# Autodesk Inventor assembly: 11_outer_carriage_with_cable_roller
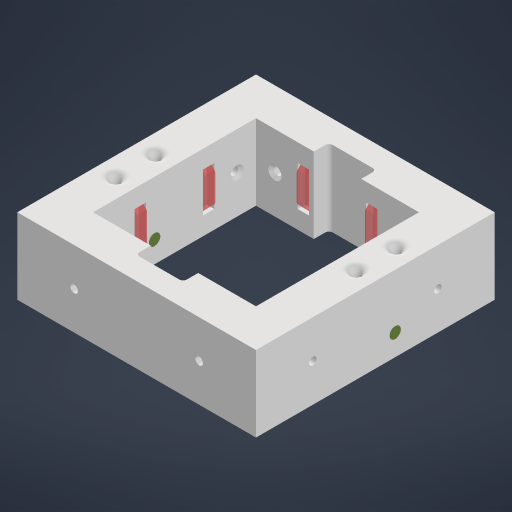
[picture p0: Inventor's stored thumbnail of the model, 512x512]
Saved by Autodesk Inventor 2024 (Build 280153000, 153)
## iProperties
Created: 2023-05-24
Part Number: 11_outer_carriage_with_cable_roller
Document SubType Name: Assembly
Designer: aasmu
Author: aasmu
## Documents named in this file (7)
- C:\Users\aasmu\Documents\standing_desk\outer_glide_carriage\11_outer_carriage_with_cable_roller.iam
- C:\Users\aasmu\Documents\standing_desk\outer_glide_carriage\02_one_side_for_cabel_roller.ipt
- C:\Users\aasmu\Documents\standing_desk\outer_glide_carriage\04_one_side_for_with_inner_cabel_pass_trough.ipt
- C:\Users\aasmu\Documents\standing_desk\inner_glide_carriage\04_steal_glide_plate.ipt
- C:\Users\aasmu\Documents\standing_desk\05_cable_roller.ipt
- C:\Users\aasmu\Documents\standing_desk\08_load_bearing.ipt
- C:\Users\aasmu\Documents\standing_desk\outer_glide_carriage\05_outer_carriage_wire_rod.ipt
## Components (20 placed, 6 different names)
1. 02_one_side_for_cabel_roller:1 — Rigid:1, Rigid:10, Rigid:11, Rigid:12, Rigid:13, Rotational:3
2. 02_one_side_for_cabel_roller:2 — Rigid:2, Rigid:3, Rigid:6, Rigid:7, Rigid:14, Rigid:15, Rotational:4
3. 04_one_side_for_with_inner_cabel_pass_trough:1 — Rigid:1, Rigid:2, Rigid:4, Rigid:5
4. 04_one_side_for_with_inner_cabel_pass_trough:2 — Rigid:3, Rigid:8, Rigid:9
5. 04_steal_glide_plate:1 — Rigid:9
6. 04_steal_glide_plate:2 — Rigid:11
7. 04_steal_glide_plate:3 — Rigid:10
8. 04_steal_glide_plate:4 — Rigid:8
9. 04_steal_glide_plate:5 — Rigid:6
10. 04_steal_glide_plate:6 — Rigid:7
11. 04_steal_glide_plate:7 — Rigid:5
12. 04_steal_glide_plate:8 — Rigid:4
13. 05_cable_roller:1 — Rotational:1
14. 05_cable_roller:2 — Rotational:2
15. 08_load_bearing:1 — Rigid:13
16. 08_load_bearing:2 — Rigid:12
17. 08_load_bearing:3 — Rigid:15
18. 08_load_bearing:4 — Rigid:14
19. 05_outer_carriage_wire_rod:1 — Rotational:1, Rotational:3
20. 05_outer_carriage_wire_rod:2 — Rotational:2, Rotational:4
## Relationships (19: WeldJoint 15, RevoluteJoint 4)
- Rigid:1 [WeldJoint]: 02_one_side_for_cabel_roller:1 ↔ 04_one_side_for_with_inner_cabel_pass_trough:1
- Rigid:2 [WeldJoint]: 02_one_side_for_cabel_roller:2 ↔ 04_one_side_for_with_inner_cabel_pass_trough:1
- Rigid:3 [WeldJoint]: 02_one_side_for_cabel_roller:2 ↔ 04_one_side_for_with_inner_cabel_pass_trough:2
- Rigid:4 [WeldJoint]: 04_one_side_for_with_inner_cabel_pass_trough:1 ↔ 04_steal_glide_plate:8
- Rigid:5 [WeldJoint]: 04_one_side_for_with_inner_cabel_pass_trough:1 ↔ 04_steal_glide_plate:7
- Rigid:6 [WeldJoint]: 02_one_side_for_cabel_roller:2 ↔ 04_steal_glide_plate:5
- Rigid:7 [WeldJoint]: 02_one_side_for_cabel_roller:2 ↔ 04_steal_glide_plate:6
- Rigid:8 [WeldJoint]: 04_one_side_for_with_inner_cabel_pass_trough:2 ↔ 04_steal_glide_plate:4
- Rigid:9 [WeldJoint]: 04_one_side_for_with_inner_cabel_pass_trough:2 ↔ 04_steal_glide_plate:1
- Rigid:10 [WeldJoint]: 02_one_side_for_cabel_roller:1 ↔ 04_steal_glide_plate:3
- Rigid:11 [WeldJoint]: 02_one_side_for_cabel_roller:1 ↔ 04_steal_glide_plate:2
- Rigid:12 [WeldJoint]: 02_one_side_for_cabel_roller:1 ↔ 08_load_bearing:2
- Rigid:13 [WeldJoint]: 02_one_side_for_cabel_roller:1 ↔ 08_load_bearing:1
- Rigid:14 [WeldJoint]: 02_one_side_for_cabel_roller:2 ↔ 08_load_bearing:4
- Rigid:15 [WeldJoint]: 02_one_side_for_cabel_roller:2 ↔ 08_load_bearing:3
- Rotational:1 [RevoluteJoint]: 05_cable_roller:1 ↔ 05_outer_carriage_wire_rod:1
- Rotational:2 [RevoluteJoint]: 05_cable_roller:2 ↔ 05_outer_carriage_wire_rod:2
- Rotational:3 [RevoluteJoint]: 02_one_side_for_cabel_roller:1 ↔ 05_outer_carriage_wire_rod:1
- Rotational:4 [RevoluteJoint]: 02_one_side_for_cabel_roller:2 ↔ 05_outer_carriage_wire_rod:2
